# Autodesk Inventor assembly: MainAssy
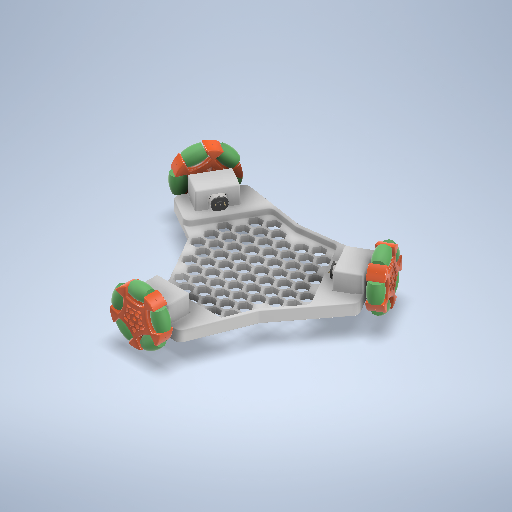
[picture p0: Inventor's stored thumbnail of the model, 512x512]
Saved by Autodesk Inventor 2025 (Build 290162000, 162)
## iProperties
Created: 2024-11-13
Part Number: MainAssy
Document SubType Name: Assembly
Designer: tvoko
Author: tvoko
## Documents named in this file (6)
- C:\Users\tvoko\Documents\Inventor\Doomba\DoombaMk1\DoombaMainAssy.iam
- C:\Users\tvoko\Documents\Inventor\Doomba\DoombaMk1\DoombaMk1Base.ipt
- C:\Users\tvoko\Documents\School\Fall 2024\Senior Design Pt 1\Lab 1\Buyouts\N20 DC MOTOR\N20 DC MOTOR.ipt
- C:\Users\tvoko\Documents\Inventor\Doomba\DoombaMk1\OmniWheels\5-Wheel 2mm Axle\5WheelAssy.iam
- C:\Users\tvoko\Documents\Inventor\Doomba\DoombaMk1\MotorMount.ipt
- C:\Users\tvoko\Documents\Inventor\Content Center Files\R2025\en-US\AS 1420\AS 1420 - 1973 - M3 x 14.ipt
## Components (16 placed, 5 different names)
1. DoombaMk1Base:1 — Mate:7, Mate:8, Mate:9, Mate:10, Mate:11, Mate:12, Mate:13, Mate:14, Mate:15, Mate:22, Mate:23, Mate:24, Mate:25, Mate:26, Mate:27, Mate:28, Mate:29, Mate:30, Mate:31, Mate:32, Mate:33
2. N20 DC MOTOR:1 — Mate:1, Mate:2, Flush:1, Mate:18, Mate:19
3. N20 DC MOTOR:2 — Mate:5, Mate:6, Flush:3, Mate:16, Mate:20
4. N20 DC MOTOR:3 — Mate:3, Flush:2, Mate:4, Mate:17, Mate:21
5. 5WheelAssy:1 [sub-assembly] — Mate:18, Mate:19
6. 5WheelAssy:2 [sub-assembly] — Mate:17, Mate:21
7. 5WheelAssy:3 [sub-assembly] — Mate:16, Mate:20
8. MotorMount:1 — Mate:5, Mate:6, Flush:3, Mate:11, Mate:12, Mate:13
9. MotorMount:2 — Mate:3, Flush:2, Mate:4, Mate:7, Mate:8, Mate:15
10. MotorMount:3 — Mate:1, Mate:2, Flush:1, Mate:9, Mate:10, Mate:14
11. AS 1420 - Metric M3 x 14:1 — Mate:23, Mate:28
12. AS 1420 - Metric M3 x 14:2 — Mate:22, Mate:29
13. AS 1420 - Metric M3 x 14:3 — Mate:26, Mate:33
14. AS 1420 - Metric M3 x 14:4 — Mate:27, Mate:32
15. AS 1420 - Metric M3 x 14:5 — Mate:24, Mate:31
16. AS 1420 - Metric M3 x 14:6 — Mate:25, Mate:30
## Relationships (36: Mate 33, Flush 3)
- Mate:1: N20 DC MOTOR:1 ↔ MotorMount:3
- Mate:2: N20 DC MOTOR:1 ↔ MotorMount:3
- Flush:1: N20 DC MOTOR:1 ↔ MotorMount:3
- Mate:3: N20 DC MOTOR:3 ↔ MotorMount:2
- Flush:2: N20 DC MOTOR:3 ↔ MotorMount:2
- Mate:4: N20 DC MOTOR:3 ↔ MotorMount:2
- Mate:5: N20 DC MOTOR:2 ↔ MotorMount:1
- Mate:6: N20 DC MOTOR:2 ↔ MotorMount:1
- Flush:3: N20 DC MOTOR:2 ↔ MotorMount:1
- Mate:7: DoombaMk1Base:1 ↔ MotorMount:2
- Mate:8: DoombaMk1Base:1 ↔ MotorMount:2
- Mate:9: DoombaMk1Base:1 ↔ MotorMount:3
- Mate:10: DoombaMk1Base:1 ↔ MotorMount:3
- Mate:11: DoombaMk1Base:1 ↔ MotorMount:1
- Mate:12: DoombaMk1Base:1 ↔ MotorMount:1
- Mate:13: DoombaMk1Base:1 ↔ MotorMount:1
- Mate:14: DoombaMk1Base:1 ↔ MotorMount:3
- Mate:15: DoombaMk1Base:1 ↔ MotorMount:2
- Mate:16: N20 DC MOTOR:2 ↔ 5WheelAssy:3
- Mate:17: N20 DC MOTOR:3 ↔ 5WheelAssy:2
- Mate:18: N20 DC MOTOR:1 ↔ 5WheelAssy:1
- Mate:19 (3 mm): N20 DC MOTOR:1 ↔ 5WheelAssy:1
- Mate:20 (3 mm): N20 DC MOTOR:2 ↔ 5WheelAssy:3
- Mate:21 (3 mm): N20 DC MOTOR:3 ↔ 5WheelAssy:2
- Mate:22: DoombaMk1Base:1 ↔ AS 1420 - Metric M3 x 14:2
- Mate:23: DoombaMk1Base:1 ↔ AS 1420 - Metric M3 x 14:1
- Mate:24: DoombaMk1Base:1 ↔ AS 1420 - Metric M3 x 14:5
- Mate:25: DoombaMk1Base:1 ↔ AS 1420 - Metric M3 x 14:6
- Mate:26: DoombaMk1Base:1 ↔ AS 1420 - Metric M3 x 14:3
- Mate:27: DoombaMk1Base:1 ↔ AS 1420 - Metric M3 x 14:4
- Mate:28: DoombaMk1Base:1 ↔ AS 1420 - Metric M3 x 14:1
- Mate:29: DoombaMk1Base:1 ↔ AS 1420 - Metric M3 x 14:2
- Mate:30: DoombaMk1Base:1 ↔ AS 1420 - Metric M3 x 14:6
- Mate:31: DoombaMk1Base:1 ↔ AS 1420 - Metric M3 x 14:5
- Mate:32: DoombaMk1Base:1 ↔ AS 1420 - Metric M3 x 14:4
- Mate:33: DoombaMk1Base:1 ↔ AS 1420 - Metric M3 x 14:3
